# Autodesk Inventor assembly: Gripper B Assembly
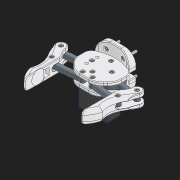
[picture p0: Inventor's stored thumbnail of the model, 180x180]
Saved by Autodesk Inventor 2017 SP1 (Build 210196100, 196)
## iProperties
Created: 2016-06-02
Part Number: Gripper B Assembly
Document SubType Name: Assembly
Designer: Zach
Sending System: SolidWorks 2013
Last Author: egomezpitarch
Last Saved: 2016-07-28
Author: Zach
## Documents named in this file (15)
- C:\Users\Zach\Documents\GitHub\BCN3D-Moveo\Autodesk Inventor files\Gripper B Assembly.iam
- C:\Users\Zach\Documents\GitHub\BCN3D-Moveo\Autodesk Inventor files\Bottom Plate C.ipt
- C:\Users\Zach\Documents\GitHub\BCN3D-Moveo\Autodesk Inventor files\Top Plate C.ipt
- C:\Users\Zach\Documents\GitHub\BCN3D-Moveo\Autodesk Inventor files\Cilinder.ipt
- C:\Users\Zach\Documents\GitHub\BCN3D-Moveo\Autodesk Inventor files\Gripper Left B.ipt
- C:\Users\Zach\Documents\GitHub\BCN3D-Moveo\Autodesk Inventor files\Gripper Right B.ipt
- C:\Users\Zach\Documents\GitHub\BCN3D-Moveo\Autodesk Inventor files\Idol Gear B.ipt
- C:\Users\Zach\Documents\GitHub\BCN3D-Moveo\Autodesk Inventor files\Pivot Arm B.ipt
- C:\Users\Zach\Documents\GitHub\BCN3D-Moveo\Autodesk Inventor files\Servo Gear B.ipt
- C:\Users\Zach\Documents\GitHub\BCN3D-Moveo\Autodesk Inventor files\M3 Nut.ipt
- C:\Users\Zach\Documents\GitHub\BCN3D-Moveo\Autodesk Inventor files\M3x16.ipt
- C:\Users\Zach\Documents\GitHub\BCN3D-Moveo\Autodesk Inventor files\M3x8.ipt
- C:\Users\Zach\Documents\GitHub\BCN3D-Moveo\Autodesk Inventor files\M3x10.ipt
- C:\Users\Zach\Documents\GitHub\tr1\lib\MG995.ipt
- C:\Users\Zach\Documents\GitHub\tr1\lib\Servo Mounting Hub.ipt
## Components (41 placed, 14 different names)
1. Bottom Plate C:1 — Mate:8, Mate:9, Mate:10, Mate:11, Mate:12, Mate:14, Mate:30, Mate:32, Mate:33, Mate:34, Mate:35, Mate:36, Mate:37, Mate:38, Mate:48, Mate:49, Mate:50, Mate:51, Mate:52, Mate:53, Angle:1
2. Top Plate C:1 — Mate:40, Mate:41, Mate:42, Mate:43, Mate:44, Mate:45, Mate:46, Mate:47, Mate:54, Mate:55, Mate:56, Mate:57, Mate:58
3. Cilinder:1
4. Gripper Left B:1 — Mate:19, Mate:21, Mate:22, Mate:24, Mate:59, Mate:60, Mate:64
5. Gripper Right B:1 — Mate:7, Mate:20, Mate:26, Mate:28, Mate:61, Mate:62, Mate:63
6. Idol Gear B:1 — Mate:1, Mate:2, Rotation:1, Mate:11, Mate:64
7. Pivot Arm B:1 — Mate:15, Mate:17, Mate:52
8. Servo Gear B:1 — Mate:4, Mate:5, Rotation:1, Mate:9, Mate:41, Mate:63, Mate:65, Mate:66, Mate:73, Mate:74, Mate:75, Mate:76
9. Pivot Arm B:2 — Mate:13, Mate:18, Mate:53
10. Cilinder:2
11. M3 Nut:1 — Mate:26, Mate:27
12. M3 Nut:5 — Mate:28, Mate:29
13. M3 Nut:6 — Mate:24, Mate:25
14. M3 Nut:7 — Mate:22, Mate:23
15. M3 Nut:8
16. M3 Nut:9
17. M3 Nut:10
18. M3 Nut:11 — Mate:30, Mate:31
19. M3 Nut:12 — Mate:38, Mate:39
20. M3x8:1 — Mate:4, Mate:10, Mate:40, Mate:43
21. M3x8:2 — Mate:74, Mate:76
22. M3x8:3 — Mate:73, Mate:75
23. M3x10:1 — Mate:36, Mate:70
24. M3x10:2 — Mate:35, Mate:69
25. M3x10:3 — Mate:34, Mate:71
26. M3x10:4 — Mate:33, Mate:72
27. M3x16:6 — Mate:1, Mate:8, Mate:57
28. M3x16:7 — Mate:31, Mate:32, Mate:58
29. M3x16:8 — Mate:37, Mate:39, Mate:55
30. M3x16:9 — Mate:12, Mate:13, Mate:42, Mate:56
31. M3x16:10 — Mate:14, Mate:15, Mate:54
32. M3x16:11 — Mate:5, Mate:7, Mate:27, Mate:62
33. M3x16:12 — Mate:2, Mate:21, Mate:23, Mate:60
34. M3x16:13 — Mate:17, Mate:20, Mate:29, Mate:61
35. M3x16:14 — Mate:18, Mate:19, Mate:25, Mate:59
36. M3x16:15 — Mate:49, Mate:50
37. M3x16:16 — Mate:48, Mate:51
38. M3x16:17 — Mate:44, Mate:47
39. M3x16:18 — Mate:45, Mate:46
40. MG995:1 — Mate:67, Mate:68, Angle:1, Mate:69, Mate:70, Mate:71, Mate:72
41. Servo Mounting Hub:1 — Mate:65, Mate:66, Mate:67, Mate:68
## Relationships (75: Mate 73, RelateRotation 1, Angle 1)
- Mate:1: Idol Gear B:1 ↔ M3x16:6
- Mate:2: Idol Gear B:1 ↔ M3x16:12
- Mate:4: Servo Gear B:1 ↔ M3x8:1
- Mate:5: Servo Gear B:1 ↔ M3x16:11
- Mate:7: Gripper Right B:1 ↔ M3x16:11
- Rotation:1 [RelateRotation] (1 ul): Idol Gear B:1 ↔ Servo Gear B:1
- Mate:8: Bottom Plate C:1 ↔ M3x16:6
- Mate:9 (0.5 mm): Bottom Plate C:1 ↔ Servo Gear B:1
- Mate:10: Bottom Plate C:1 ↔ M3x8:1
- Mate:11 (0.5 mm): Bottom Plate C:1 ↔ Idol Gear B:1
- Mate:12: Bottom Plate C:1 ↔ M3x16:9
- Mate:13: Pivot Arm B:2 ↔ M3x16:9
- Mate:14: Bottom Plate C:1 ↔ M3x16:10
- Mate:15: Pivot Arm B:1 ↔ M3x16:10
- Mate:17: Pivot Arm B:1 ↔ M3x16:13
- Mate:18: Pivot Arm B:2 ↔ M3x16:14
- Mate:19: Gripper Left B:1 ↔ M3x16:14
- Mate:20: Gripper Right B:1 ↔ M3x16:13
- Mate:21: Gripper Left B:1 ↔ M3x16:12
- Mate:22: Gripper Left B:1 ↔ M3 Nut:7
- Mate:23: M3 Nut:7 ↔ M3x16:12
- Mate:24: Gripper Left B:1 ↔ M3 Nut:6
- Mate:25: M3 Nut:6 ↔ M3x16:14
- Mate:26: Gripper Right B:1 ↔ M3 Nut:1
- Mate:27: M3 Nut:1 ↔ M3x16:11
- Mate:28: Gripper Right B:1 ↔ M3 Nut:5
- Mate:29: M3 Nut:5 ↔ M3x16:13
- Mate:30: Bottom Plate C:1 ↔ M3 Nut:11
- Mate:31: M3 Nut:11 ↔ M3x16:7
- Mate:32: Bottom Plate C:1 ↔ M3x16:7
- Mate:33: Bottom Plate C:1 ↔ M3x10:4
- Mate:34: Bottom Plate C:1 ↔ M3x10:3
- Mate:35: Bottom Plate C:1 ↔ M3x10:2
- Mate:36: Bottom Plate C:1 ↔ M3x10:1
- Mate:37: Bottom Plate C:1 ↔ M3x16:8
- Mate:38: Bottom Plate C:1 ↔ M3 Nut:12
- Mate:39: M3 Nut:12 ↔ M3x16:8
- Mate:40: Top Plate C:1 ↔ M3x8:1
- Mate:41 (0.5 mm): Top Plate C:1 ↔ Servo Gear B:1
- Mate:42: Top Plate C:1 ↔ M3x16:9
- Mate:43: Top Plate C:1 ↔ M3x8:1
- Mate:44: Top Plate C:1 ↔ M3x16:17
- Mate:45: Top Plate C:1 ↔ M3x16:18
- Mate:46: Top Plate C:1 ↔ M3x16:18
- Mate:47: Top Plate C:1 ↔ M3x16:17
- Mate:48: Bottom Plate C:1 ↔ M3x16:16
- Mate:49: Bottom Plate C:1 ↔ M3x16:15
- Mate:50: Bottom Plate C:1 ↔ M3x16:15
- Mate:51: Bottom Plate C:1 ↔ M3x16:16
- Mate:52 (0.5 mm): Bottom Plate C:1 ↔ Pivot Arm B:1
- Mate:53 (0.5 mm): Bottom Plate C:1 ↔ Pivot Arm B:2
- Mate:54: Top Plate C:1 ↔ M3x16:10
- Mate:55: Top Plate C:1 ↔ M3x16:8
- Mate:56: Top Plate C:1 ↔ M3x16:9
- Mate:57: Top Plate C:1 ↔ M3x16:6
- Mate:58: Top Plate C:1 ↔ M3x16:7
- Mate:59: Gripper Left B:1 ↔ M3x16:14
- Mate:60: Gripper Left B:1 ↔ M3x16:12
- Mate:61: Gripper Right B:1 ↔ M3x16:13
- Mate:62: Gripper Right B:1 ↔ M3x16:11
- Mate:63 (0.5 mm): Gripper Right B:1 ↔ Servo Gear B:1
- Mate:64 (0.5 mm): Gripper Left B:1 ↔ Idol Gear B:1
- Mate:65: Servo Gear B:1 ↔ Servo Mounting Hub:1
- Mate:66: Servo Gear B:1 ↔ Servo Mounting Hub:1
- Mate:67: MG995:1 ↔ Servo Mounting Hub:1
- Mate:68: MG995:1 ↔ Servo Mounting Hub:1
- Angle:1 (0 deg): Bottom Plate C:1 ↔ MG995:1
- Mate:69: M3x10:2 ↔ MG995:1
- Mate:70: M3x10:1 ↔ MG995:1
- Mate:71: M3x10:3 ↔ MG995:1
- Mate:72: M3x10:4 ↔ MG995:1
- Mate:73: Servo Gear B:1 ↔ M3x8:3
- Mate:74: Servo Gear B:1 ↔ M3x8:2
- Mate:75: Servo Gear B:1 ↔ M3x8:3
- Mate:76: Servo Gear B:1 ↔ M3x8:2
